# Autodesk Inventor assembly: Robot Base Complete Darkmatter
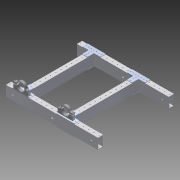
[picture p0: Inventor's stored thumbnail of the model, 180x180]
Saved by Autodesk Inventor 2015 (Build 190159000, 159)
## iProperties
Created: 2014-12-20
Part Number: Robot Base Complete Darkmatter
Document SubType Name: Assembly
Designer: Nemo
Author: Nemo
## Documents named in this file (5)
- U:\Robot Base Complete Darkmatter.iam
- U:\26x30 Frame\VersaFrame End Rail 12-20-14.ipt
- U:\26x30 Frame\VersaFrame Side Rail 12-20-14.ipt
- U:\COTS Parts\VersaFrame\VersaFrame VersaChassis Gusset.ipt
- U:\Tetrix motor mount.ipt
## Components (14 placed, 6 different names)
1. VersaFrame End Rail: Front — Mate:1, Flush:1, Flush:2, Flush:3, Flush:8, Flush:9, Mate:6, Flush:14, Mate:7, Flush:16, Flush:18, Flush:19, Mate:9, Mate:11, Flush:22, Mate:12, Flush:24
2. VersaFrame End Rail: Back — Mate:1, Flush:2, Mate:4, Flush:10, Mate:5, Flush:13, Mate:10, Mate:13, Flush:27, Mate:14, Flush:29, Flush:30, Flush:31
3. VersaFrame Side Rail: Right — Flush:18, Mate:8, Flush:19, Flush:20, Flush:21, Flush:25, Flush:28
4. VersaFrame Side Rail: Left — Flush:7, Flush:8, Flush:9, Flush:12, Flush:17, Mate:9, Mate:10, Flush:23, Flush:26
5. Tetrix motor mount:1 — Flush:31, Mate:16, Flush:32
6. Tetrix motor mount:2 — Flush:30, Mate:15
7. VersaFrame VersaChassis Gusset:1 — Mate:7, Flush:16, Flush:17
8. VersaFrame VersaChassis Gusset:2 — Mate:6, Flush:14, Flush:20
9. VersaFrame VersaChassis Gusset:3 — Mate:5, Flush:12, Flush:13
10. VersaFrame VersaChassis Gusset:4 — Mate:4, Flush:10, Flush:21
11. VersaFrame VersaChassis Gusset:5 — Mate:11, Flush:22, Flush:23
12. VersaFrame VersaChassis Gusset:6 — Mate:12, Flush:24, Flush:25
13. VersaFrame VersaChassis Gusset:7 — Mate:13, Flush:26, Flush:27, Mate:16, Flush:32
14. VersaFrame VersaChassis Gusset:8 — Mate:14, Flush:28, Flush:29, Mate:15
## Relationships (41: Flush 27, Mate 14)
- Mate:1: VersaFrame End Rail: Front ↔ VersaFrame End Rail: Back
- Flush:1 (52.3875 mm): VersaFrame End Rail: Front
- Flush:2: VersaFrame End Rail: Front ↔ VersaFrame End Rail: Back
- Flush:3: VersaFrame End Rail: Front
- Flush:7: VersaFrame Side Rail: Left
- Flush:8: VersaFrame End Rail: Front ↔ VersaFrame Side Rail: Left
- Flush:9 (146.05 mm): VersaFrame End Rail: Front ↔ VersaFrame Side Rail: Left
- Mate:4: VersaFrame End Rail: Back ↔ VersaFrame VersaChassis Gusset:4
- Flush:10: VersaFrame End Rail: Back ↔ VersaFrame VersaChassis Gusset:4
- Mate:5: VersaFrame End Rail: Back ↔ VersaFrame VersaChassis Gusset:3
- Flush:12: VersaFrame Side Rail: Left ↔ VersaFrame VersaChassis Gusset:3
- Flush:13: VersaFrame End Rail: Back ↔ VersaFrame VersaChassis Gusset:3
- Mate:6: VersaFrame End Rail: Front ↔ VersaFrame VersaChassis Gusset:2
- Flush:14: VersaFrame End Rail: Front ↔ VersaFrame VersaChassis Gusset:2
- Mate:7: VersaFrame End Rail: Front ↔ VersaFrame VersaChassis Gusset:1
- Flush:16: VersaFrame End Rail: Front ↔ VersaFrame VersaChassis Gusset:1
- Flush:17: VersaFrame Side Rail: Left ↔ VersaFrame VersaChassis Gusset:1
- Flush:18: VersaFrame End Rail: Front ↔ VersaFrame Side Rail: Right
- Mate:8: VersaFrame Side Rail: Right
- Flush:19 (57.15 mm): VersaFrame End Rail: Front ↔ VersaFrame Side Rail: Right
- Mate:9: VersaFrame End Rail: Front ↔ VersaFrame Side Rail: Left
- Mate:10: VersaFrame End Rail: Back ↔ VersaFrame Side Rail: Left
- Flush:20: VersaFrame Side Rail: Right ↔ VersaFrame VersaChassis Gusset:2
- Flush:21: VersaFrame Side Rail: Right ↔ VersaFrame VersaChassis Gusset:4
- Mate:11: VersaFrame End Rail: Front ↔ VersaFrame VersaChassis Gusset:5
- Flush:22: VersaFrame End Rail: Front ↔ VersaFrame VersaChassis Gusset:5
- Flush:23: VersaFrame Side Rail: Left ↔ VersaFrame VersaChassis Gusset:5
- Mate:12: VersaFrame End Rail: Front ↔ VersaFrame VersaChassis Gusset:6
- Flush:24: VersaFrame End Rail: Front ↔ VersaFrame VersaChassis Gusset:6
- Flush:25: VersaFrame Side Rail: Right ↔ VersaFrame VersaChassis Gusset:6
- Mate:13: VersaFrame End Rail: Back ↔ VersaFrame VersaChassis Gusset:7
- Flush:26: VersaFrame Side Rail: Left ↔ VersaFrame VersaChassis Gusset:7
- Flush:27: VersaFrame End Rail: Back ↔ VersaFrame VersaChassis Gusset:7
- Mate:14: VersaFrame End Rail: Back ↔ VersaFrame VersaChassis Gusset:8
- Flush:28: VersaFrame Side Rail: Right ↔ VersaFrame VersaChassis Gusset:8
- Flush:29: VersaFrame End Rail: Back ↔ VersaFrame VersaChassis Gusset:8
- Flush:30: VersaFrame End Rail: Back ↔ Tetrix motor mount:2
- Mate:15: Tetrix motor mount:2 ↔ VersaFrame VersaChassis Gusset:8
- Flush:31 (6.35 mm): VersaFrame End Rail: Back ↔ Tetrix motor mount:1
- Mate:16: Tetrix motor mount:1 ↔ VersaFrame VersaChassis Gusset:7
- Flush:32 (-14.7828 mm): Tetrix motor mount:1 ↔ VersaFrame VersaChassis Gusset:7
## Named parameters: SideRailOffset = 50.8 mm, CenterDrop = 3.175 mm
